# Autodesk Inventor assembly: !Chassis-fixed
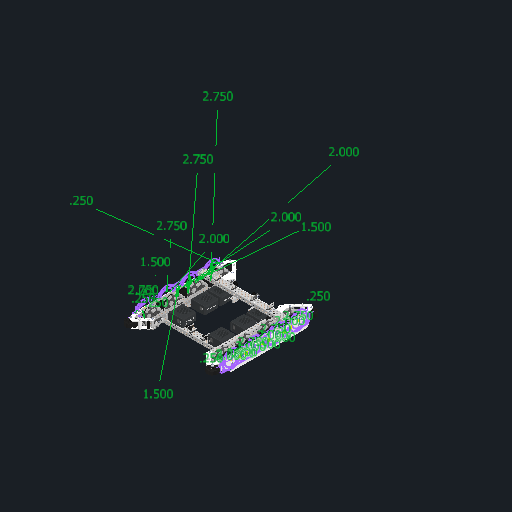
[picture p0: Inventor's stored thumbnail of the model, 512x512]
Saved by Autodesk Inventor 2025.1 (Build 291241020, 241B)
## iProperties
Created: 2024-12-27
Part Number: !Chassis-fixed
Document SubType Name: Assembly
Designer: Averey Ku
Author: Averey Ku
## Documents named in this file (5)
- C:\Users\peter\VEX\High Stakes\CAD\V4\Chassis\!Chassis-fixed.iam
- C:\Users\peter\VEX\High Stakes\CAD\V4\Chassis\Crossbrace\!Crossbrace.iam
- C:\Users\peter\VEX\High Stakes\CAD\V4\Chassis\Drivebay Left\!Drivebay Left.iam
- C:\Users\peter\VEX\High Stakes\CAD\V4\Chassis\Drivebay Right\!Drivebay Right.iam
- C:\Users\peter\VEX\High Stakes\CAD\V4\Chassis\Ramp\!Ramp.iam
## Components (4 placed, 4 different names)
1. !Crossbrace:1 [sub-assembly] — Insert:1, Mate:1, Insert:2, Mate:2
2. !Drivebay Left:1 [sub-assembly] — Insert:1, Mate:1, Insert:3
3. !Drivebay Right:1 [sub-assembly] — Insert:2, Mate:2, Mate:3
4. !Ramp:1 [sub-assembly] — Insert:3, Mate:3
## Relationships (6: Insert 3, Mate 3)
- Insert:1: !Crossbrace:1 ↔ !Drivebay Left:1
- Mate:1: !Crossbrace:1 ↔ !Drivebay Left:1
- Insert:2: !Crossbrace:1 ↔ !Drivebay Right:1
- Mate:2: !Crossbrace:1 ↔ !Drivebay Right:1
- Insert:3: !Drivebay Left:1 ↔ !Ramp:1
- Mate:3: !Drivebay Right:1 ↔ !Ramp:1
